# Autodesk Inventor assembly: nhk1_1
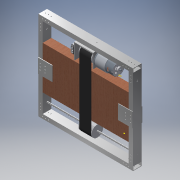
[picture p0: Inventor's stored thumbnail of the model, 180x180]
Saved by Autodesk Inventor 2019 (Build 230136000, 136)
## iProperties
Created: 2022-02-15
Part Number: nhk1_1
Material: 一般
Document SubType Name: Assembly
Designer: yuta
Author: yuta
## Documents named in this file (14)
- C:\Users\yuta\Documents\キャチロボ\nhk1_1.iam
- C:\Users\yuta\Documents\キャチロボ\nhk11.ipt
- C:\Users\yuta\Documents\キャチロボ\nhk13.ipt
- C:\Users\yuta\Documents\キャチロボ\RS775_CAD_IAM\モーター RS775-8513DF.iam
- C:\Users\yuta\Documents\キャチロボ\nhk14.ipt
- C:\Users\yuta\Documents\キャチロボ\nhk16.ipt
- C:\Users\yuta\Documents\キャチロボ\amt102-v-1.snapshot.2\AMT-B0-W.ipt
- C:\Users\yuta\Documents\キャチロボ\amt102-v-1.snapshot.2\amt102-v.iam
- C:\Users\yuta\Documents\キャチロボ\nhk17.ipt
- C:\Users\yuta\Documents\キャチロボ\nhk15.ipt
- C:\Users\yuta\Documents\キャチロボ\nhk18.ipt
- C:\Users\yuta\Documents\キャチロボ\nhk20.ipt
- C:\Users\yuta\Documents\キャチロボ\nhk19.ipt
- C:\Users\yuta\Documents\キャチロボ\nhk21.ipt
## Components (18 placed, 13 different names)
1. nhk11:1 — メイト:1, メイト:2, メイト:3, メイト:4, メイト:7, メイト:8
2. nhk13:1 — メイト:1, メイト:2, メイト:5
3. nhk13:2 — メイト:3, メイト:4
4. モーター RS775-8513DF:1 [sub-assembly] — メイト:5, メイト:6
5. nhk14:1 — メイト:6, メイト:7, メイト:9, メイト:10
6. nhk16:1 — メイト:9, メイト:10, メイト:11, メイト:12, メイト:14, メイト:15, メイト:16
7. AMT-B0-W:1 — メイト:11, メイト:12, メイト:13
8. amt102-v:2 [sub-assembly] — メイト:13, メイト:14
9. nhk17:1 — メイト:15, メイト:16, メイト:17, メイト:18, メイト:19, メイト:20, メイト:21, メイト:22
10. nhk15:1 — メイト:23, メイト:24, メイト:25
11. nhk18:1 — メイト:17, メイト:18, メイト:19, メイト:26, メイト:27, メイト:28
12. nhk18:2 — メイト:20, メイト:21, メイト:22, メイト:23, メイト:24, メイト:25, メイト:30, メイト:31, メイト:36, フラッシュ:1
13. nhk20:1 — メイト:30, メイト:31, メイト:32
14. nhk20:2 — メイト:34, メイト:35
15. nhk20:3 — メイト:26, メイト:27, メイト:29
16. nhk20:4 — メイト:28, メイト:29, メイト:33
17. nhk19:1 — メイト:32, メイト:33, メイト:34, メイト:35
18. nhk21:1 — メイト:36, フラッシュ:1
## Relationships (37: Mate 36, Flush 1)
- メイト:1 [Mate]: nhk11:1 ↔ nhk13:1
- メイト:2 [Mate]: nhk11:1 ↔ nhk13:1
- メイト:3 [Mate]: nhk11:1 ↔ nhk13:2
- メイト:4 [Mate]: nhk11:1 ↔ nhk13:2
- メイト:5 [Mate]: nhk13:1 ↔ モーター RS775-8513DF:1
- メイト:6 [Mate]: モーター RS775-8513DF:1 ↔ nhk14:1
- メイト:7 [Mate]: nhk11:1 ↔ nhk14:1
- メイト:8 [Mate]: nhk11:1
- メイト:9 [Mate]: nhk14:1 ↔ nhk16:1
- メイト:10 [Mate]: nhk14:1 ↔ nhk16:1
- メイト:11 [Mate]: nhk16:1 ↔ AMT-B0-W:1
- メイト:12 [Mate]: nhk16:1 ↔ AMT-B0-W:1
- メイト:13 [Mate]: AMT-B0-W:1 ↔ amt102-v:2
- メイト:14 [Mate]: nhk16:1 ↔ amt102-v:2
- メイト:15 [Mate]: nhk16:1 ↔ nhk17:1
- メイト:16 [Mate]: nhk16:1 ↔ nhk17:1
- メイト:17 [Mate]: nhk17:1 ↔ nhk18:1
- メイト:18 [Mate]: nhk17:1 ↔ nhk18:1
- メイト:19 [Mate]: nhk17:1 ↔ nhk18:1
- メイト:20 [Mate]: nhk17:1 ↔ nhk18:2
- メイト:21 [Mate]: nhk17:1 ↔ nhk18:2
- メイト:22 [Mate]: nhk17:1 ↔ nhk18:2
- メイト:23 [Mate]: nhk15:1 ↔ nhk18:2
- メイト:24 [Mate]: nhk15:1 ↔ nhk18:2
- メイト:25 [Mate]: nhk15:1 ↔ nhk18:2
- メイト:26 [Mate]: nhk18:1 ↔ nhk20:3
- メイト:27 [Mate]: nhk18:1 ↔ nhk20:3
- メイト:28 [Mate]: nhk18:1 ↔ nhk20:4
- メイト:29 [Mate]: nhk20:3 ↔ nhk20:4
- メイト:30 [Mate]: nhk18:2 ↔ nhk20:1
- メイト:31 [Mate]: nhk18:2 ↔ nhk20:1
- メイト:32 [Mate]: nhk20:1 ↔ nhk19:1
- メイト:33 [Mate]: nhk20:4 ↔ nhk19:1
- メイト:34 [Mate]: nhk20:2 ↔ nhk19:1
- メイト:35 [Mate]: nhk20:2 ↔ nhk19:1
- メイト:36 [Mate]: nhk18:2 ↔ nhk21:1
- フラッシュ:1 [Flush]: nhk18:2 ↔ nhk21:1
